# Autodesk Inventor assembly: Assembly1
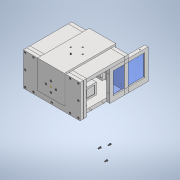
[picture p0: Inventor's stored thumbnail of the model, 180x180]
Saved by Autodesk Inventor 2022.2 (Build 262287030, 287C)
## iProperties
Created: 2022-01-28
Part Number: Assembly1
Document SubType Name: Assembly
Designer: Tapendra
Author: Tapendra
## Documents named in this file (30)
- C:\Users\Tapendra\Documents\opticalbox\Assembly1.iam
- C:\Users\Tapendra\Documents\opticalbox\base.ipt
- C:\Users\Tapendra\Documents\opticalbox\back.ipt
- C:\Users\Tapendra\Documents\opticalbox\top.ipt
- C:\Users\Tapendra\Documents\opticalbox\leftright.ipt
- C:\Users\Tapendra\Documents\opticalbox\CCM1-BS013.ipt
- C:\Users\Tapendra\Documents\opticalbox\front.ipt
- C:\Users\Tapendra\Documents\opticalbox\topwindow.ipt
- C:\Users\Tapendra\Documents\opticalbox\acrylicpmt.ipt
- C:\Users\Tapendra\Documents\opticalbox\toppmt.ipt
- C:\Users\Tapendra\Documents\opticalbox\left.ipt
- C:\Users\Tapendra\Documents\opticalbox\SM1D12-Step.ipt
- C:\Users\Tapendra\Documents\opticalbox\ELL14K-Step.ipt
- C:\Users\Tapendra\Documents\opticalbox\CFC11P-A-Step.ipt
- C:\Users\Tapendra\Documents\opticalbox\WP25M-UB-Step.ipt
- C:\Users\Tapendra\Documents\opticalbox\92078A216_Polycarbonate Dowel Pin.ipt
- C:\Users\Tapendra\Documents\opticalbox\baseblock.ipt
- C:\Users\Tapendra\Documents\opticalbox\baseplate.ipt
- C:\Users\Tapendra\Documents\opticalbox\MOT1102_0_3D.iam
- C:\Users\Tapendra\Documents\opticalbox\sidebracket.ipt
- C:\Users\Tapendra\Documents\opticalbox\pmtholder.ipt
- C:\Users\Tapendra\Documents\opticalbox\pmtbase.ipt
- C:\Users\Tapendra\Documents\Inventor\Content Center Files\R2022\en-US\UNI EN ISO 7045  H\EN ISO 7045 - M2 x  6 - 4.8 - H.ipt
- C:\Users\Tapendra\Documents\opticalbox\acrylicwindow.ipt
- C:\Users\Tapendra\Documents\opticalbox\93365A120_Tapered Heat-Set Inserts for Plastic.ipt
- C:\Users\Tapendra\Documents\Inventor\Content Center Files\R2022\en-US\AS 1427(01)\AS 1427 - M3 x 12(3).ipt
- C:\Users\Tapendra\Documents\Inventor\Content Center Files\R2022\en-US\AS 1427(01)\AS 1427 - M3 x 8(3).ipt
- C:\Users\Tapendra\Documents\Inventor\Content Center Files\R2022\en-US\AS 1427(11)\AS 1427 - M3 x 8(8).ipt
- C:\Users\Tapendra\Documents\opticalbox\92185A105_Super-Corrosion-Resistant 316 Stainless Steel Socket Head Screw.ipt
- C:\Users\Tapendra\Documents\opticalbox\93615A110_18-8 Stainless Steel Low-Profile Socket Head Screw.ipt
## Components (122 placed, 29 different names)
1. base:1 — Mate:1, Flush:1, Flush:2, Flush:8, Flush:9, Mate:15, Mate:24, Mate:25, Mate:26, Mate:27, Mate:33, Mate:34, Mate:35, Mate:57, Mate:60, Mate:61, Mate:64, Mate:86, Mate:92, Mate:144, Mate:145, Mate:146, Mate:147, Mate:148, Mate:149, Mate:150, Mate:151, Mate:153, Mate:154, Insert:20, Insert:21, Insert:22, Insert:23, Insert:24, Insert:25
2. back:1 — Mate:1, Flush:1, Flush:2, Mate:2, Flush:3, Flush:4, Mate:7, Mate:13, Mate:36, Mate:37, Mate:38, Mate:39, Mate:50, Mate:51, Mate:55, Mate:56, Mate:66, Mate:68, Mate:81, Mate:82, Mate:83, Mate:84, Mate:125, Mate:126, Mate:141, Mate:142
3. top:1 — Mate:2, Flush:3, Flush:4, Mate:5, Flush:6, Mate:6, Flush:7, Mate:73, Mate:74, Mate:75, Mate:76, Mate:77, Mate:78, Mate:79, Mate:80, Insert:5, Insert:34, Insert:35, Insert:36, Insert:37, Insert:38, Insert:39, Insert:40, Insert:41, Insert:42, Insert:43, Insert:44
4. front:1 — Mate:5, Flush:6, Mate:40, Mate:41, Mate:42, Mate:43, Mate:44, Mate:45, Mate:46, Mate:47, Mate:48, Mate:52, Mate:53, Mate:54, Mate:69, Mate:70, Mate:71, Mate:72, Mate:143
5. topwindow:1 — Mate:6, Flush:7, Insert:16, Insert:17, Insert:18, Insert:19, Insert:45, Insert:46, Insert:47, Insert:48, Insert:49, Insert:50, Insert:51, Insert:52, Insert:53, Insert:54, Insert:55, Insert:56
6. acrylicpmt:1 — Mate:85
7. leftright:1 — Mate:7, Flush:8, Mate:85, Mate:157, Mate:158, Mate:159
8. toppmt:1 — Mate:139, Mate:140
9. left:1 — Mate:13, Flush:9, Mate:86, Mate:143
10. CFC11P-A-Step:1 — Mate:30
11. ELL14K-Step:1 — Insert:1, Mate:22, Mate:23, Mate:30
12. WP25M-UB-Step:1 — Insert:1
13. CCM1-BS013:2 — Mate:17, Mate:18, Mate:22, Mate:23, Mate:87, Mate:88, Mate:122, Mate:152, Mate:160, Mate:161, Mate:162, Mate:163
14. 92078A216_Polycarbonate Dowel Pin:1 — Mate:40, Mate:41
15. 92078A216_Polycarbonate Dowel Pin:2 — Mate:26, Mate:27
16. 92078A216_Polycarbonate Dowel Pin:3 — Mate:15, Mate:33
17. 92078A216_Polycarbonate Dowel Pin:4 — Mate:144, Mate:145
18. 92078A216_Polycarbonate Dowel Pin:5 — Mate:34, Mate:35
19. 92078A216_Polycarbonate Dowel Pin:6 — Mate:146, Mate:147
20. 92078A216_Polycarbonate Dowel Pin:7 — Mate:24, Mate:25
21. 92078A216_Polycarbonate Dowel Pin:8 — Mate:38, Mate:39
22. 92078A216_Polycarbonate Dowel Pin:9 — Mate:36, Mate:37
23. SM1D12-Step:1 — Mate:17, Mate:18, Mate:121
24. 92078A216_Polycarbonate Dowel Pin:10 — Mate:53, Mate:54
25. 92078A216_Polycarbonate Dowel Pin:12 — Mate:60, Mate:61
26. 92078A216_Polycarbonate Dowel Pin:13 — Mate:42, Mate:43
27. 92078A216_Polycarbonate Dowel Pin:14 — Mate:50, Mate:56
28. 92078A216_Polycarbonate Dowel Pin:15 — Mate:44, Mate:45
29. 92078A216_Polycarbonate Dowel Pin:16 — Mate:46, Mate:47
30. 92078A216_Polycarbonate Dowel Pin:17 — Mate:48, Mate:52
31. 92078A216_Polycarbonate Dowel Pin:18 — Mate:148, Mate:149
32. 92078A216_Polycarbonate Dowel Pin:19 — Mate:57, Mate:64
33. 92078A216_Polycarbonate Dowel Pin:20 — Mate:150, Mate:151
34. 92078A216_Polycarbonate Dowel Pin:21 — Mate:141, Mate:142
35. 92078A216_Polycarbonate Dowel Pin:22 — Mate:66, Mate:68
36. 92078A216_Polycarbonate Dowel Pin:25 — Mate:51, Mate:55
37. 92078A216_Polycarbonate Dowel Pin:26 — Mate:75, Mate:77
38. 92078A216_Polycarbonate Dowel Pin:27 — Mate:70, Mate:71
39. 92078A216_Polycarbonate Dowel Pin:28 — Mate:74, Mate:79
40. 92078A216_Polycarbonate Dowel Pin:29 — Mate:76, Mate:78
41. 92078A216_Polycarbonate Dowel Pin:30 — Mate:73, Mate:80
42. 92078A216_Polycarbonate Dowel Pin:31 — Mate:81, Mate:82
43. 92078A216_Polycarbonate Dowel Pin:32 — Mate:69, Mate:72
44. 92078A216_Polycarbonate Dowel Pin:36 — Mate:83, Mate:84
45. baseblock:1 — Flush:91, Mate:90, Mate:91, Mate:92, Mate:153, Mate:154, Insert:26, Insert:27
46. baseplate:1 — Mate:87, Mate:88, Mate:89, Mate:91, Insert:28, Insert:29
47. 92078A216_Polycarbonate Dowel Pin:37 — Mate:89, Flush:91, Mate:90
48. MOT1102_0_3D:1 [sub-assembly]
49. sidebracket:1 — Mate:125, Mate:126, Insert:57, Insert:58, Insert:59, Insert:60, Insert:61, Insert:62, Insert:63, Insert:64, Insert:73
50. pmtholder:1 — Mate:123, Mate:124, Mate:164, Insert:69, Insert:70, Insert:71, Insert:72
51. pmtbase:1 — Mate:121, Mate:122, Mate:123, Mate:124, Mate:139, Mate:140, Mate:152, Insert:3, Mate:155, Insert:4, Mate:156, Insert:8, Insert:9, Insert:10, Insert:11, Insert:30, Insert:31, Insert:32, Insert:33, Mate:164
52. UNI EN ISO 7045 H M2 x  6 - 4.8 - H:1 — Mate:155
53. UNI EN ISO 7045 H M2 x  6 - 4.8 - H:2 — Mate:156
54. UNI EN ISO 7045 H M2 x  6 - 4.8 - H:3 — Insert:4
55. UNI EN ISO 7045 H M2 x  6 - 4.8 - H:4 — Insert:3
56. acrylicwindow:1 — Mate:157, Mate:158, Mate:159
57. 93365A120_Tapered Heat-Set Inserts for Plastic:1 — Insert:17
58. 93365A120_Tapered Heat-Set Inserts for Plastic:2 — Insert:16
59. 93365A120_Tapered Heat-Set Inserts for Plastic:3 — Insert:19
60. 93365A120_Tapered Heat-Set Inserts for Plastic:4 — Insert:21
61. 93365A120_Tapered Heat-Set Inserts for Plastic:5 — Insert:9
62. 93365A120_Tapered Heat-Set Inserts for Plastic:6 — Insert:11
63. 93365A120_Tapered Heat-Set Inserts for Plastic:7 — Insert:10
64. 93365A120_Tapered Heat-Set Inserts for Plastic:8 — Insert:8
65. 93365A120_Tapered Heat-Set Inserts for Plastic:9 — Insert:5
66. 93365A120_Tapered Heat-Set Inserts for Plastic:10 — Insert:18
67. 93365A120_Tapered Heat-Set Inserts for Plastic:11 — Insert:20
68. 93365A120_Tapered Heat-Set Inserts for Plastic:12 — Insert:22
69. 93365A120_Tapered Heat-Set Inserts for Plastic:15 — Insert:23
70. 93365A120_Tapered Heat-Set Inserts for Plastic:16 — Insert:43
71. 93365A120_Tapered Heat-Set Inserts for Plastic:20 — Insert:36
72. 93365A120_Tapered Heat-Set Inserts for Plastic:21 — Insert:37
73. 93365A120_Tapered Heat-Set Inserts for Plastic:22 — Insert:35
74. 93365A120_Tapered Heat-Set Inserts for Plastic:23 — Insert:39
75. 93365A120_Tapered Heat-Set Inserts for Plastic:24 — Insert:32
76. 93365A120_Tapered Heat-Set Inserts for Plastic:25 — Insert:34
77. 93365A120_Tapered Heat-Set Inserts for Plastic:26 — Insert:24
78. 93365A120_Tapered Heat-Set Inserts for Plastic:27 — Insert:25
79. 93365A120_Tapered Heat-Set Inserts for Plastic:28 — Insert:31
80. 93365A120_Tapered Heat-Set Inserts for Plastic:29 — Insert:38
81. 93365A120_Tapered Heat-Set Inserts for Plastic:30 — Insert:40
82. 93365A120_Tapered Heat-Set Inserts for Plastic:31 — Insert:44
83. 93365A120_Tapered Heat-Set Inserts for Plastic:32 — Insert:41
84. 93365A120_Tapered Heat-Set Inserts for Plastic:33 — Insert:42
85. 93365A120_Tapered Heat-Set Inserts for Plastic:34 — Insert:30
86. 93365A120_Tapered Heat-Set Inserts for Plastic:35 — Insert:33
87. AS 1427 - Metric M3 x 12:11 — Insert:26
88. AS 1427 - Metric M3 x 12:12 — Insert:27
89. AS 1427 - Metric M3 x 8:6 — Insert:28
90. AS 1427 - Metric M3 x 8:7 — Insert:29
91. AS 1427 Raised - Metric M3 x 8:1 — Mate:160
92. AS 1427 Raised - Metric M3 x 8:2 — Mate:161
93. AS 1427 Raised - Metric M3 x 8:3 — Mate:163
94. AS 1427 Raised - Metric M3 x 8:4 — Mate:162
95. AS 1427 - Metric M3 x 12:13 — Insert:47
96. AS 1427 - Metric M3 x 12:14 — Insert:48
97. AS 1427 - Metric M3 x 12:15 — Insert:45
98. AS 1427 - Metric M3 x 12:16 — Insert:46
99. AS 1427 - Metric M3 x 12:17 — Insert:49
100. AS 1427 - Metric M3 x 12:18 — Insert:50
101. AS 1427 - Metric M3 x 12:19 — Insert:51
102. AS 1427 - Metric M3 x 12:20 — Insert:52
103. AS 1427 - Metric M3 x 12:21 — Insert:53
104. AS 1427 - Metric M3 x 12:22 — Insert:54
105. AS 1427 - Metric M3 x 12:23 — Insert:56
106. AS 1427 - Metric M3 x 12:24 — Insert:55
107. AS 1427 - Metric M3 x 8:8 — Insert:62
108. AS 1427 - Metric M3 x 8:9 — Insert:57
109. AS 1427 - Metric M3 x 8:10 — Insert:60
110. AS 1427 - Metric M3 x 8:11 — Insert:61
111. AS 1427 - Metric M3 x 8:12 — Insert:64
112. AS 1427 - Metric M3 x 8:13 — Insert:63
113. AS 1427 - Metric M3 x 8:14 — Insert:59
114. AS 1427 - Metric M3 x 8:15 — Insert:58
115. 92185A105_Super-Corrosion-Resistant 316 Stainless Steel Socket Head Screw:1 — Insert:69
116. 92185A105_Super-Corrosion-Resistant 316 Stainless Steel Socket Head Screw:2 — Insert:72
117. 92185A105_Super-Corrosion-Resistant 316 Stainless Steel Socket Head Screw:3 — Insert:71
118. 92185A105_Super-Corrosion-Resistant 316 Stainless Steel Socket Head Screw:4 — Insert:70
119. 93615A110_18-8 Stainless Steel Low-Profile Socket Head Screw:1
120. 93615A110_18-8 Stainless Steel Low-Profile Socket Head Screw:2 — Insert:73
121. 93615A110_18-8 Stainless Steel Low-Profile Socket Head Screw:3
122. 93615A110_18-8 Stainless Steel Low-Profile Socket Head Screw:4
## Relationships (172: Mate 101, Insert 62, Flush 9)
- Mate:1: base:1 ↔ back:1
- Flush:1: base:1 ↔ back:1
- Flush:2: base:1 ↔ back:1
- Mate:2: back:1 ↔ top:1
- Flush:3: back:1 ↔ top:1
- Flush:4: back:1 ↔ top:1
- Mate:5: top:1 ↔ front:1
- Flush:6: top:1 ↔ front:1
- Mate:6: top:1 ↔ topwindow:1
- Flush:7: top:1 ↔ topwindow:1
- Mate:7: back:1 ↔ leftright:1
- Flush:8: base:1 ↔ leftright:1
- Mate:13: back:1 ↔ left:1
- Flush:9: base:1 ↔ left:1
- Insert:1 (-10 mm): ELL14K-Step:1 ↔ WP25M-UB-Step:1
- Mate:15: base:1 ↔ 92078A216_Polycarbonate Dowel Pin:3
- Mate:17: CCM1-BS013:2 ↔ SM1D12-Step:1
- Mate:18: CCM1-BS013:2 ↔ SM1D12-Step:1
- Mate:22: ELL14K-Step:1 ↔ CCM1-BS013:2
- Mate:23: ELL14K-Step:1 ↔ CCM1-BS013:2
- Mate:24: base:1 ↔ 92078A216_Polycarbonate Dowel Pin:7
- Mate:25: base:1 ↔ 92078A216_Polycarbonate Dowel Pin:7
- Mate:26: base:1 ↔ 92078A216_Polycarbonate Dowel Pin:2
- Mate:27: base:1 ↔ 92078A216_Polycarbonate Dowel Pin:2
- Mate:30: CFC11P-A-Step:1 ↔ ELL14K-Step:1
- Mate:33: base:1 ↔ 92078A216_Polycarbonate Dowel Pin:3
- Mate:34: base:1 ↔ 92078A216_Polycarbonate Dowel Pin:5
- Mate:35: base:1 ↔ 92078A216_Polycarbonate Dowel Pin:5
- Mate:36: back:1 ↔ 92078A216_Polycarbonate Dowel Pin:9
- Mate:37: back:1 ↔ 92078A216_Polycarbonate Dowel Pin:9
- Mate:38: back:1 ↔ 92078A216_Polycarbonate Dowel Pin:8
- Mate:39: back:1 ↔ 92078A216_Polycarbonate Dowel Pin:8
- Mate:40: front:1 ↔ 92078A216_Polycarbonate Dowel Pin:1
- Mate:41: front:1 ↔ 92078A216_Polycarbonate Dowel Pin:1
- Mate:42: front:1 ↔ 92078A216_Polycarbonate Dowel Pin:13
- Mate:43: front:1 ↔ 92078A216_Polycarbonate Dowel Pin:13
- Mate:44: front:1 ↔ 92078A216_Polycarbonate Dowel Pin:15
- Mate:45: front:1 ↔ 92078A216_Polycarbonate Dowel Pin:15
- Mate:46: front:1 ↔ 92078A216_Polycarbonate Dowel Pin:16
- Mate:47: front:1 ↔ 92078A216_Polycarbonate Dowel Pin:16
- Mate:48: front:1 ↔ 92078A216_Polycarbonate Dowel Pin:17
- Mate:50: back:1 ↔ 92078A216_Polycarbonate Dowel Pin:14
- Mate:51: back:1 ↔ 92078A216_Polycarbonate Dowel Pin:25
- Mate:52: front:1 ↔ 92078A216_Polycarbonate Dowel Pin:17
- Mate:53: front:1 ↔ 92078A216_Polycarbonate Dowel Pin:10
- Mate:54: front:1 ↔ 92078A216_Polycarbonate Dowel Pin:10
- Mate:55: back:1 ↔ 92078A216_Polycarbonate Dowel Pin:25
- Mate:56: back:1 ↔ 92078A216_Polycarbonate Dowel Pin:14
- Mate:57: base:1 ↔ 92078A216_Polycarbonate Dowel Pin:19
- Mate:60: base:1 ↔ 92078A216_Polycarbonate Dowel Pin:12
- Mate:61: base:1 ↔ 92078A216_Polycarbonate Dowel Pin:12
- Mate:64: base:1 ↔ 92078A216_Polycarbonate Dowel Pin:19
- Mate:66: back:1 ↔ 92078A216_Polycarbonate Dowel Pin:22
- Mate:68: back:1 ↔ 92078A216_Polycarbonate Dowel Pin:22
- Mate:69: front:1 ↔ 92078A216_Polycarbonate Dowel Pin:32
- Mate:70: front:1 ↔ 92078A216_Polycarbonate Dowel Pin:27
- Mate:71: front:1 ↔ 92078A216_Polycarbonate Dowel Pin:27
- Mate:72: front:1 ↔ 92078A216_Polycarbonate Dowel Pin:32
- Mate:73: top:1 ↔ 92078A216_Polycarbonate Dowel Pin:30
- Mate:74: top:1 ↔ 92078A216_Polycarbonate Dowel Pin:28
- Mate:75: top:1 ↔ 92078A216_Polycarbonate Dowel Pin:26
- Mate:76: top:1 ↔ 92078A216_Polycarbonate Dowel Pin:29
- Mate:77: top:1 ↔ 92078A216_Polycarbonate Dowel Pin:26
- Mate:78: top:1 ↔ 92078A216_Polycarbonate Dowel Pin:29
- Mate:79: top:1 ↔ 92078A216_Polycarbonate Dowel Pin:28
- Mate:80: top:1 ↔ 92078A216_Polycarbonate Dowel Pin:30
- Mate:81: back:1 ↔ 92078A216_Polycarbonate Dowel Pin:31
- Mate:82: back:1 ↔ 92078A216_Polycarbonate Dowel Pin:31
- Mate:83: back:1 ↔ 92078A216_Polycarbonate Dowel Pin:36
- Mate:84: back:1 ↔ 92078A216_Polycarbonate Dowel Pin:36
- Mate:85: acrylicpmt:1 ↔ leftright:1
- Mate:86: base:1 ↔ left:1
- Mate:87: CCM1-BS013:2 ↔ baseplate:1
- Mate:88: CCM1-BS013:2 ↔ baseplate:1
- Mate:89: baseplate:1 ↔ 92078A216_Polycarbonate Dowel Pin:37
- Flush:91: baseblock:1 ↔ 92078A216_Polycarbonate Dowel Pin:37
- Mate:90: baseblock:1 ↔ 92078A216_Polycarbonate Dowel Pin:37
- Mate:91: baseblock:1 ↔ baseplate:1
- Mate:92: base:1 ↔ baseblock:1
- Mate:121: SM1D12-Step:1 ↔ pmtbase:1
- Mate:122: CCM1-BS013:2 ↔ pmtbase:1
- Mate:123: pmtholder:1 ↔ pmtbase:1
- Mate:124: pmtholder:1 ↔ pmtbase:1
- Mate:125: back:1 ↔ sidebracket:1
- Mate:126 (20 mm): back:1 ↔ sidebracket:1
- Mate:139: toppmt:1 ↔ pmtbase:1
- Mate:140: toppmt:1 ↔ pmtbase:1
- Mate:141: back:1 ↔ 92078A216_Polycarbonate Dowel Pin:21
- Mate:142: back:1 ↔ 92078A216_Polycarbonate Dowel Pin:21
- Mate:143: front:1 ↔ left:1
- Mate:144: base:1 ↔ 92078A216_Polycarbonate Dowel Pin:4
- Mate:145: base:1 ↔ 92078A216_Polycarbonate Dowel Pin:4
- Mate:146: base:1 ↔ 92078A216_Polycarbonate Dowel Pin:6
- Mate:147: base:1 ↔ 92078A216_Polycarbonate Dowel Pin:6
- Mate:148: base:1 ↔ 92078A216_Polycarbonate Dowel Pin:18
- Mate:149: base:1 ↔ 92078A216_Polycarbonate Dowel Pin:18
- Mate:150: base:1 ↔ 92078A216_Polycarbonate Dowel Pin:20
- Mate:151: base:1 ↔ 92078A216_Polycarbonate Dowel Pin:20
- Mate:152: CCM1-BS013:2 ↔ pmtbase:1
- Mate:153: base:1 ↔ baseblock:1
- Mate:154: base:1 ↔ baseblock:1
- Insert:3: pmtbase:1 ↔ UNI EN ISO 7045 H M2 x  6 - 4.8 - H:4
- Mate:155: pmtbase:1 ↔ UNI EN ISO 7045 H M2 x  6 - 4.8 - H:1
- Insert:4: pmtbase:1 ↔ UNI EN ISO 7045 H M2 x  6 - 4.8 - H:3
- Mate:156: pmtbase:1 ↔ UNI EN ISO 7045 H M2 x  6 - 4.8 - H:2
- Mate:157: leftright:1 ↔ acrylicwindow:1
- Mate:158: leftright:1 ↔ acrylicwindow:1
- Mate:159: leftright:1 ↔ acrylicwindow:1
- Insert:5: top:1 ↔ 93365A120_Tapered Heat-Set Inserts for Plastic:9
- Insert:8: pmtbase:1 ↔ 93365A120_Tapered Heat-Set Inserts for Plastic:8
- Insert:9: pmtbase:1 ↔ 93365A120_Tapered Heat-Set Inserts for Plastic:5
- Insert:10: pmtbase:1 ↔ 93365A120_Tapered Heat-Set Inserts for Plastic:7
- Insert:11: pmtbase:1 ↔ 93365A120_Tapered Heat-Set Inserts for Plastic:6
- Insert:16: topwindow:1 ↔ 93365A120_Tapered Heat-Set Inserts for Plastic:2
- Insert:17: topwindow:1 ↔ 93365A120_Tapered Heat-Set Inserts for Plastic:1
- Insert:18: topwindow:1 ↔ 93365A120_Tapered Heat-Set Inserts for Plastic:10
- Insert:19: topwindow:1 ↔ 93365A120_Tapered Heat-Set Inserts for Plastic:3
- Insert:20: base:1 ↔ 93365A120_Tapered Heat-Set Inserts for Plastic:11
- Insert:21: base:1 ↔ 93365A120_Tapered Heat-Set Inserts for Plastic:4
- Insert:22: base:1 ↔ 93365A120_Tapered Heat-Set Inserts for Plastic:12
- Insert:23: base:1 ↔ 93365A120_Tapered Heat-Set Inserts for Plastic:15
- Insert:24: base:1 ↔ 93365A120_Tapered Heat-Set Inserts for Plastic:26
- Insert:25: base:1 ↔ 93365A120_Tapered Heat-Set Inserts for Plastic:27
- Insert:26: baseblock:1 ↔ AS 1427 - Metric M3 x 12:11
- Insert:27: baseblock:1 ↔ AS 1427 - Metric M3 x 12:12
- Insert:28: baseplate:1 ↔ AS 1427 - Metric M3 x 8:6
- Insert:29: baseplate:1 ↔ AS 1427 - Metric M3 x 8:7
- Mate:160: CCM1-BS013:2 ↔ AS 1427 Raised - Metric M3 x 8:1
- Mate:161: CCM1-BS013:2 ↔ AS 1427 Raised - Metric M3 x 8:2
- Mate:162: CCM1-BS013:2 ↔ AS 1427 Raised - Metric M3 x 8:4
- Mate:163: CCM1-BS013:2 ↔ AS 1427 Raised - Metric M3 x 8:3
- Insert:30: pmtbase:1 ↔ 93365A120_Tapered Heat-Set Inserts for Plastic:34
- Insert:31: pmtbase:1 ↔ 93365A120_Tapered Heat-Set Inserts for Plastic:28
- Insert:32: pmtbase:1 ↔ 93365A120_Tapered Heat-Set Inserts for Plastic:24
- Insert:33: pmtbase:1 ↔ 93365A120_Tapered Heat-Set Inserts for Plastic:35
- Mate:164: pmtholder:1 ↔ pmtbase:1
- Insert:34: top:1 ↔ 93365A120_Tapered Heat-Set Inserts for Plastic:25
- Insert:35: top:1 ↔ 93365A120_Tapered Heat-Set Inserts for Plastic:22
- Insert:36: top:1 ↔ 93365A120_Tapered Heat-Set Inserts for Plastic:20
- Insert:37: top:1 ↔ 93365A120_Tapered Heat-Set Inserts for Plastic:21
- Insert:38: top:1 ↔ 93365A120_Tapered Heat-Set Inserts for Plastic:29
- Insert:39: top:1 ↔ 93365A120_Tapered Heat-Set Inserts for Plastic:23
- Insert:40: top:1 ↔ 93365A120_Tapered Heat-Set Inserts for Plastic:30
- Insert:41: top:1 ↔ 93365A120_Tapered Heat-Set Inserts for Plastic:32
- Insert:42: top:1 ↔ 93365A120_Tapered Heat-Set Inserts for Plastic:33
- Insert:43: top:1 ↔ 93365A120_Tapered Heat-Set Inserts for Plastic:16
- Insert:44: top:1 ↔ 93365A120_Tapered Heat-Set Inserts for Plastic:31
- Insert:45: topwindow:1 ↔ AS 1427 - Metric M3 x 12:15
- Insert:46: topwindow:1 ↔ AS 1427 - Metric M3 x 12:16
- Insert:47: topwindow:1 ↔ AS 1427 - Metric M3 x 12:13
- Insert:48: topwindow:1 ↔ AS 1427 - Metric M3 x 12:14
- Insert:49: topwindow:1 ↔ AS 1427 - Metric M3 x 12:17
- Insert:50: topwindow:1 ↔ AS 1427 - Metric M3 x 12:18
- Insert:51: topwindow:1 ↔ AS 1427 - Metric M3 x 12:19
- Insert:52: topwindow:1 ↔ AS 1427 - Metric M3 x 12:20
- Insert:53: topwindow:1 ↔ AS 1427 - Metric M3 x 12:21
- Insert:54: topwindow:1 ↔ AS 1427 - Metric M3 x 12:22
- Insert:55: topwindow:1 ↔ AS 1427 - Metric M3 x 12:24
- Insert:56: topwindow:1 ↔ AS 1427 - Metric M3 x 12:23
- Insert:57: sidebracket:1 ↔ AS 1427 - Metric M3 x 8:9
- Insert:58: sidebracket:1 ↔ AS 1427 - Metric M3 x 8:15
- Insert:59: sidebracket:1 ↔ AS 1427 - Metric M3 x 8:14
- Insert:60: sidebracket:1 ↔ AS 1427 - Metric M3 x 8:10
- Insert:61: sidebracket:1 ↔ AS 1427 - Metric M3 x 8:11
- Insert:62: sidebracket:1 ↔ AS 1427 - Metric M3 x 8:8
- Insert:63: sidebracket:1 ↔ AS 1427 - Metric M3 x 8:13
- Insert:64: sidebracket:1 ↔ AS 1427 - Metric M3 x 8:12
- Insert:69: pmtholder:1 ↔ 92185A105_Super-Corrosion-Resistant 316 Stainless Steel Socket Head Screw:1
- Insert:70: pmtholder:1 ↔ 92185A105_Super-Corrosion-Resistant 316 Stainless Steel Socket Head Screw:4
- Insert:71: pmtholder:1 ↔ 92185A105_Super-Corrosion-Resistant 316 Stainless Steel Socket Head Screw:3
- Insert:72: pmtholder:1 ↔ 92185A105_Super-Corrosion-Resistant 316 Stainless Steel Socket Head Screw:2
- Insert:73: sidebracket:1 ↔ 93615A110_18-8 Stainless Steel Low-Profile Socket Head Screw:2
